# Autodesk Inventor assembly: Throughput Mockup Assembly v1p1
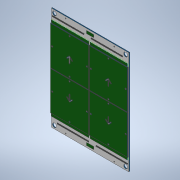
[picture p0: Inventor's stored thumbnail of the model, 180x180]
Saved by Autodesk Inventor 2022 (Build 260153000, 153)
## iProperties
Created: 2022-05-17
Part Number: Throughput Mockup Assembly v1p1
Document SubType Name: Assembly
Designer: Caleb
Author: Caleb
## iProperties of the stored document etl_module_pcb_mockup_v3p1.ipt
Created: 2022-05-17
Part Number: etl_module_pcb_mockup_v3p1
Material: Generic
Description: FreeCAD Model
Document SubType Name: Modeling
Designer: Caleb
Authority: Unknown
Density: 1 g/cm^3
Appearance: Default
Sending System: FreeCAD
Preprocessor: Open CASCADE STEP processor 7.5
Title: Open CASCADE Shape Model
Author: Author
## Documents named in this file (4)
- C:\Users\Caleb\Desktop\nebraska-silicon-lab\Hardware\ETL\modules\throughput mockups\Throughput Mockup Assembly v1p1.iam
- **C:\Users\Caleb\Desktop\nebraska-silicon-lab\Hardware\ETL\modules\throughput mockups\Throughput Mockup Assembly v1p1.iam*LocalDocs*xAaaaqrdaAaaaaaaaAaaaq1cc4b*etl_module_pcb_mockup_v3p1.ipt
- C:\Users\Caleb\Desktop\nebraska-silicon-lab\Hardware\ETL\modules\throughput mockups\BBM Assembly v1p1.iam
- C:\Users\Caleb\Desktop\nebraska-silicon-lab\Hardware\ETL\modules\throughput mockups\etl_module_pcb_mockup_v3p1.step
## Components (5 placed, 2 different names)
1. etl_module_pcb_mockup_v3p1:1 — Mate:1, Mate:2, Mate:3, Mate:4, Angle:1, Angle:2, Angle:3
2. BBM Assembly v1p1:1 [sub-assembly] — Mate:2, Angle:1, Mate:5, Flush:1, Flush:2, Mate:6
3. BBM Assembly v1p1:2 [sub-assembly] — Mate:1, Mate:5, Flush:1, Flush:3
4. BBM Assembly v1p1:3 [sub-assembly] — Mate:3, Angle:2, Flush:2, Flush:4, Mate:6
5. BBM Assembly v1p1:4 [sub-assembly] — Mate:4, Angle:3, Flush:3, Flush:4
## Relationships (13: Mate 6, Flush 4, Angle 3)
- Mate:1: etl_module_pcb_mockup_v3p1:1 ↔ BBM Assembly v1p1:2
- Mate:2: etl_module_pcb_mockup_v3p1:1 ↔ BBM Assembly v1p1:1
- Mate:3: etl_module_pcb_mockup_v3p1:1 ↔ BBM Assembly v1p1:3
- Mate:4: etl_module_pcb_mockup_v3p1:1 ↔ BBM Assembly v1p1:4
- Angle:1 (0 deg): etl_module_pcb_mockup_v3p1:1 ↔ BBM Assembly v1p1:1
- Angle:2 (0 deg): etl_module_pcb_mockup_v3p1:1 ↔ BBM Assembly v1p1:3
- Angle:3 (0 deg): etl_module_pcb_mockup_v3p1:1 ↔ BBM Assembly v1p1:4
- Mate:5 (0.2 mm): BBM Assembly v1p1:1 ↔ BBM Assembly v1p1:2
- Flush:1: BBM Assembly v1p1:1 ↔ BBM Assembly v1p1:2
- Flush:2: BBM Assembly v1p1:1 ↔ BBM Assembly v1p1:3
- Flush:3: BBM Assembly v1p1:2 ↔ BBM Assembly v1p1:4
- Flush:4: BBM Assembly v1p1:3 ↔ BBM Assembly v1p1:4
- Mate:6 (0.2 mm): BBM Assembly v1p1:1 ↔ BBM Assembly v1p1:3
